# Autodesk Inventor assembly: Krzyżakiam
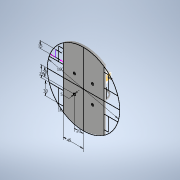
[picture p0: Inventor's stored thumbnail of the model, 180x180]
Saved by Autodesk Inventor 2020 (Build 240168000, 168)
## iProperties
Created: 2023-01-12
Part Number: Krzyżakiam
Document SubType Name: Assembly
Designer: User
Author: User
## Documents named in this file (8)
- C:\Users\User\Documents\Inventor\Krzyżakiam.iam
- C:\Users\User\Documents\Inventor\platforma wriertnicza.ipt
- C:\Users\User\Documents\Inventor\heheheha.ipt
- C:\Users\User\Documents\Inventor\prent1.ipt
- C:\Users\User\Documents\Inventor\Silnik.ipt
- D:\inventor\Silnik_MIR.ipt
- C:\Users\User\Documents\Inventor\wzrok.ipt
- C:\Users\User\Documents\Inventor\łapka.ipt
## Components (12 placed, 7 different names)
1. platforma wriertnicza:1 — Wstawiające:6, Wstawiające:7, Zestawiające:2, Zestawiające:3, Zestawiające:4, Wstawiające:8, Wstawiające:9, Wstawiające:10, Wstawiające:11
2. heheheha:1 — Wstawiające:2, Wstawiające:3, Wstawiające:4, Wstawiające:5, Zestawiające:1, Równoległe:1
3. prent1:1 — Wstawiające:2
4. prent1:2 — Wstawiające:3, Wstawiające:6
5. prent1:4 — Wstawiające:4, Wstawiające:7
6. prent1:5 — Wstawiające:5
7. Silnik:1 — Zestawiające:1, Równoległe:1, Równoległe:2
8. Silnik_MIR:1 — Równoległe:2
9. wzrok:1 — Wstawiające:8
10. wzrok:2 — Zestawiające:2, Zestawiające:3, Zestawiające:4
11. wzrok:3 — Wstawiające:9
12. łapka:1 — Wstawiające:10, Wstawiające:11
## Relationships (16: Insert 10, Mate 4, Flush 2)
- Wstawiające:2 [Insert]: heheheha:1 ↔ prent1:1
- Wstawiające:3 [Insert]: heheheha:1 ↔ prent1:2
- Wstawiające:4 [Insert]: heheheha:1 ↔ prent1:4
- Wstawiające:5 [Insert]: heheheha:1 ↔ prent1:5
- Wstawiające:6 [Insert]: platforma wriertnicza:1 ↔ prent1:2
- Wstawiające:7 [Insert]: platforma wriertnicza:1 ↔ prent1:4
- Zestawiające:1 [Mate]: heheheha:1 ↔ Silnik:1
- Równoległe:1 [Flush]: heheheha:1 ↔ Silnik:1
- Równoległe:2 [Flush]: Silnik:1 ↔ Silnik_MIR:1
- Zestawiające:2 [Mate]: platforma wriertnicza:1 ↔ wzrok:2
- Zestawiające:3 [Mate]: platforma wriertnicza:1 ↔ wzrok:2
- Zestawiające:4 [Mate] (2 mm): platforma wriertnicza:1 ↔ wzrok:2
- Wstawiające:8 [Insert] (2 mm): platforma wriertnicza:1 ↔ wzrok:1
- Wstawiające:9 [Insert] (2 mm): platforma wriertnicza:1 ↔ wzrok:3
- Wstawiające:10 [Insert]: platforma wriertnicza:1 ↔ łapka:1
- Wstawiające:11 [Insert]: platforma wriertnicza:1 ↔ łapka:1
